# Autodesk Inventor assembly: upper_arm
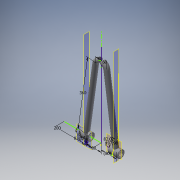
[picture p0: Inventor's stored thumbnail of the model, 180x180]
Saved by Autodesk Inventor 2016 SP1 (Build 200210100, 210)
## iProperties
Created: 2016-06-15
Part Number: upper_arm
Document SubType Name: Assembly
Designer: asvsf
Author: asvsf
## Documents named in this file (5)
- C:\Project\Buggy\Suspension\upper_arm.iam
- C:\Project\Buggy\Suspension\upper_arm_001.ipt
- C:\Project\Buggy\Suspension\upper_arm_004.ipt
- C:\Project\Buggy\Suspension\upper_arm\Design Accelerator\Bearing1.iam
- C:\Project\Buggy\Suspension\upper_arm_005.ipt
## Components (8 placed, 4 different names)
1. upper_arm_001:1 — Tangent:2, Mate:21, Tangent:3, Mate:24, Angle:1, Angle:2, Mate:26
2. upper_arm_004:3 — Flush:7, Mate:19, Flush:8, Mate:20, Tangent:2, Angle:1
3. Bearing:3 [sub-assembly] — Flush:7, Mate:19
4. Bearing:4 [sub-assembly] — Flush:8, Mate:20
5. upper_arm_004:4 — Mate:22, Flush:9, Mate:23, Flush:10, Tangent:3, Mate:24, Angle:2
6. Bearing:5 [sub-assembly] — Mate:22, Flush:9
7. Bearing:6 [sub-assembly] — Mate:23, Flush:10
8. upper_arm_005:1 — Mate:26
## Relationships (15: Mate 7, Flush 4, Tangent 2, Angle 2)
- Flush:7: upper_arm_004:3 ↔ Bearing:3
- Mate:19: upper_arm_004:3 ↔ Bearing:3
- Flush:8: upper_arm_004:3 ↔ Bearing:4
- Mate:20: upper_arm_004:3 ↔ Bearing:4
- Tangent:2: upper_arm_001:1 ↔ upper_arm_004:3
- Mate:21: upper_arm_001:1
- Mate:22: upper_arm_004:4 ↔ Bearing:5
- Flush:9: upper_arm_004:4 ↔ Bearing:5
- Mate:23: upper_arm_004:4 ↔ Bearing:6
- Flush:10: upper_arm_004:4 ↔ Bearing:6
- Tangent:3: upper_arm_001:1 ↔ upper_arm_004:4
- Mate:24: upper_arm_001:1 ↔ upper_arm_004:4
- Angle:1 (0 deg): upper_arm_001:1 ↔ upper_arm_004:3
- Angle:2 (0 deg): upper_arm_001:1 ↔ upper_arm_004:4
- Mate:26: upper_arm_001:1 ↔ upper_arm_005:1
